# Autodesk Inventor assembly: Assembly_Cube_Kinematic_Mirrormount_Astromedia_30x40x1_45_PRO_magnetic
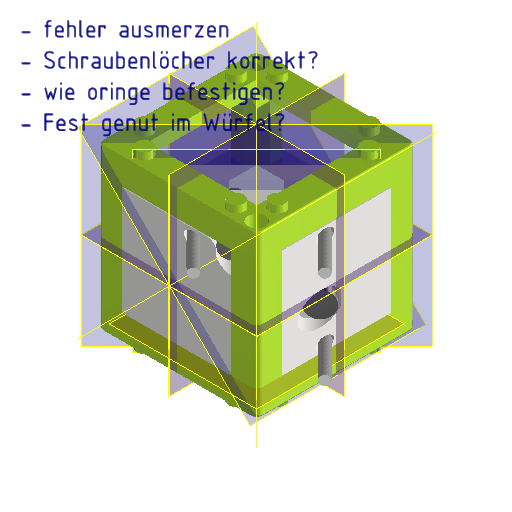
[picture p0: Inventor's stored thumbnail of the model, 512x512]
Saved by Autodesk Inventor 2022 (Build 260153000, 153)
## iProperties
Created: 2021-11-15
Part Number: Assembly_Cube_Kinematic_Mirrormount_Astromedia_30x40x1_45_PRO_magnetic
Document SubType Name: Assembly
Designer: diederichbenedict
Author: diederichbenedict
## Documents named in this file (9)
- C:\Users\diederichbenedict\Dropbox\Dokumente\Promotion\PROJECTS\openUC2-CAD\INVENTOR\Assembly_Cube_Kinematic_Mirrormount_Astromedia_30x40x1_45_PRO_magnetic.iam
- C:\Users\diederichbenedict\Dropbox\Dokumente\Promotion\PROJECTS\openUC2-CAD\INVENTOR\Assembly_Cube_empty_IM_v3.iam
- C:\Users\diederichbenedict\Dropbox\Dokumente\Promotion\PROJECTS\openUC2-CAD\INVENTOR\00_Astromedia_FronSurfaceMirror_40x30mmx1mm.ipt
- C:\Users\diederichbenedict\Dropbox\Dokumente\Promotion\PROJECTS\openUC2-CAD\INVENTOR\content\DIN 914\DIN 914 - M3 x 20.ipt
- C:\Users\diederichbenedict\Dropbox\Dokumente\Promotion\PROJECTS\openUC2-CAD\INVENTOR\20_Cube_Insert_Kinematic_Astromedia_30x40x1_45_pro_magnetic.ipt
- C:\Users\diederichbenedict\Dropbox\Dokumente\Promotion\PROJECTS\openUC2-CAD\INVENTOR\20_Cube_Insert_Kinematic_Mirror_45_pro_magnetic.ipt
- C:\Users\diederichbenedict\Dropbox\Dokumente\Promotion\PROJECTS\openUC2-CAD\INVENTOR\00_NeoDymMagnet_8x3mm.ipt
- C:\Users\diederichbenedict\Dropbox\Dokumente\Promotion\PROJECTS\openUC2-CAD\INVENTOR\00_Screw_Ball_Spring_Head_M3x30mm.ipt
- C:\Users\diederichbenedict\Dropbox\Dokumente\Promotion\PROJECTS\openUC2-CAD\INVENTOR\00_Threaded_Screw_Insert_M3.ipt
## Components (15 placed, 8 different names)
1. Assembly_Cube_empty_IM_v3:1 [sub-assembly] — Fluchtend:1, Fluchtend:2, Fluchtend:3, Fluchtend:4, Fluchtend:5, Passend:1, Passend:2
2. 20_Cube_Insert_Kinematic_Mirror_45_pro_magnetic:1 — Fluchtend:1, Fluchtend:2, Fluchtend:4, Fluchtend:5, Einfügen:9, Einfügen:10, Einfügen:13, Einfügen:14, Einfügen:15
3. 20_Cube_Insert_Kinematic_Astromedia_30x40x1_45_pro_magnetic:1 — Fluchtend:3, Passend:1, Passend:2, Passend:3, Einfügen:11, Einfügen:12
4. 00_Astromedia_FronSurfaceMirror_40x30mmx1mm:1 — Passend:3
5. DIN 914 M3 x 20:4
6. 00_NeoDymMagnet_8x3mm:1 — Einfügen:10
7. 00_NeoDymMagnet_8x3mm:2 — Einfügen:9
8. 00_NeoDymMagnet_8x3mm:3 — Einfügen:12
9. 00_NeoDymMagnet_8x3mm:4 — Einfügen:11
10. 00_Screw_Ball_Spring_Head_M3x30mm:1 — Einfügen:16
11. 00_Threaded_Screw_Insert_M3:1 — Einfügen:13, Einfügen:17
12. 00_Threaded_Screw_Insert_M3:2 — Einfügen:15, Einfügen:18
13. 00_Threaded_Screw_Insert_M3:3 — Einfügen:14, Einfügen:16
14. 00_Screw_Ball_Spring_Head_M3x30mm:2 — Einfügen:17
15. 00_Screw_Ball_Spring_Head_M3x30mm:3 — Einfügen:18
## Relationships (18: Insert 10, Flush 5, Mate 3)
- Fluchtend:1 [Flush]: Assembly_Cube_empty_IM_v3:1 ↔ 20_Cube_Insert_Kinematic_Mirror_45_pro_magnetic:1
- Fluchtend:2 [Flush]: Assembly_Cube_empty_IM_v3:1 ↔ 20_Cube_Insert_Kinematic_Mirror_45_pro_magnetic:1
- Fluchtend:3 [Flush]: Assembly_Cube_empty_IM_v3:1 ↔ 20_Cube_Insert_Kinematic_Astromedia_30x40x1_45_pro_magnetic:1
- Fluchtend:4 [Flush]: Assembly_Cube_empty_IM_v3:1 ↔ 20_Cube_Insert_Kinematic_Mirror_45_pro_magnetic:1
- Fluchtend:5 [Flush]: Assembly_Cube_empty_IM_v3:1 ↔ 20_Cube_Insert_Kinematic_Mirror_45_pro_magnetic:1
- Passend:1 [Mate]: Assembly_Cube_empty_IM_v3:1 ↔ 20_Cube_Insert_Kinematic_Astromedia_30x40x1_45_pro_magnetic:1
- Passend:2 [Mate]: Assembly_Cube_empty_IM_v3:1 ↔ 20_Cube_Insert_Kinematic_Astromedia_30x40x1_45_pro_magnetic:1
- Passend:3 [Mate] (-1 mm): 20_Cube_Insert_Kinematic_Astromedia_30x40x1_45_pro_magnetic:1 ↔ 00_Astromedia_FronSurfaceMirror_40x30mmx1mm:1
- Einfügen:9 [Insert]: 20_Cube_Insert_Kinematic_Mirror_45_pro_magnetic:1 ↔ 00_NeoDymMagnet_8x3mm:2
- Einfügen:10 [Insert]: 20_Cube_Insert_Kinematic_Mirror_45_pro_magnetic:1 ↔ 00_NeoDymMagnet_8x3mm:1
- Einfügen:11 [Insert]: 20_Cube_Insert_Kinematic_Astromedia_30x40x1_45_pro_magnetic:1 ↔ 00_NeoDymMagnet_8x3mm:4
- Einfügen:12 [Insert]: 20_Cube_Insert_Kinematic_Astromedia_30x40x1_45_pro_magnetic:1 ↔ 00_NeoDymMagnet_8x3mm:3
- Einfügen:13 [Insert]: 20_Cube_Insert_Kinematic_Mirror_45_pro_magnetic:1 ↔ 00_Threaded_Screw_Insert_M3:1
- Einfügen:14 [Insert]: 20_Cube_Insert_Kinematic_Mirror_45_pro_magnetic:1 ↔ 00_Threaded_Screw_Insert_M3:3
- Einfügen:15 [Insert]: 20_Cube_Insert_Kinematic_Mirror_45_pro_magnetic:1 ↔ 00_Threaded_Screw_Insert_M3:2
- Einfügen:16 [Insert] (-10 mm): 00_Screw_Ball_Spring_Head_M3x30mm:1 ↔ 00_Threaded_Screw_Insert_M3:3
- Einfügen:17 [Insert] (-10 mm): 00_Threaded_Screw_Insert_M3:1 ↔ 00_Screw_Ball_Spring_Head_M3x30mm:2
- Einfügen:18 [Insert] (-10 mm): 00_Threaded_Screw_Insert_M3:2 ↔ 00_Screw_Ball_Spring_Head_M3x30mm:3
